# Autodesk Inventor assembly: Platform assembly
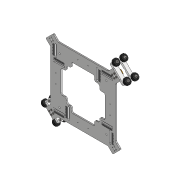
[picture p0: Inventor's stored thumbnail of the model, 180x180]
Saved by Autodesk Inventor 2020 (Build 240168000, 168)
## iProperties
Created: 2020-12-15
Part Number: Platform assembly
Document SubType Name: Assembly
Designer: ferrerx
Author: ferrerx
## Documents named in this file (4)
- C:\Users\ferrerx\Desktop\Prieto-Godino Lab\Drosophila Larvae Behavioural Device\Device design V3\Inventor Assembly\Platform assembly.iam
- C:\Users\ferrerx\Desktop\Prieto-Godino Lab\Drosophila Larvae Behavioural Device\Device design V3\Inventor Assembly\Light sources platform.ipt
- C:\Users\ferrerx\Desktop\Prieto-Godino Lab\Drosophila Larvae Behavioural Device\Device design V3\Inventor Assembly\Cart assembly.iam
- C:\Users\ferrerx\Documents\Inventor\Content Center Files\R2020\en-US\AS 1427(05)\AS 1427 - M3 x 25(5) II.ipt
## Components (11 placed, 3 different names)
1. Light sources platform:1 — Mate:1, Mate:2, Angle:1, Mate:3, Mate:4, Angle:2, Mate:6, Mate:7, Mate:8, Mate:9, Mate:10, Mate:11, Mate:12, Mate:13, Mate:14, Mate:15, Mate:16, Mate:17, Mate:18, Mate:19, Mate:20
2. Cart assembly:1 [sub-assembly] — Mate:1, Mate:2, Angle:1, Mate:5
3. Cart assembly:2 [sub-assembly] — Mate:3, Mate:4, Angle:2
4. AS 1427 H - Metric M3 x 25:1 — Mate:5, Mate:6
5. AS 1427 H - Metric M3 x 25:2 — Mate:7, Mate:19
6. AS 1427 H - Metric M3 x 25:3 — Mate:9, Mate:20
7. AS 1427 H - Metric M3 x 25:4 — Mate:8, Mate:18
8. AS 1427 H - Metric M3 x 25:5 — Mate:12, Mate:16
9. AS 1427 H - Metric M3 x 25:6 — Mate:10, Mate:17
10. AS 1427 H - Metric M3 x 25:7 — Mate:13, Mate:14
11. AS 1427 H - Metric M3 x 25:8 — Mate:11, Mate:15
## Relationships (22: Mate 20, Angle 2)
- Mate:1: Light sources platform:1 ↔ Cart assembly:1
- Mate:2: Light sources platform:1 ↔ Cart assembly:1
- Angle:1 (0 deg): Light sources platform:1 ↔ Cart assembly:1
- Mate:3: Light sources platform:1 ↔ Cart assembly:2
- Mate:4: Light sources platform:1 ↔ Cart assembly:2
- Angle:2 (0 deg): Light sources platform:1 ↔ Cart assembly:2
- Mate:5: Cart assembly:1 ↔ AS 1427 H - Metric M3 x 25:1
- Mate:6: Light sources platform:1 ↔ AS 1427 H - Metric M3 x 25:1
- Mate:7: Light sources platform:1 ↔ AS 1427 H - Metric M3 x 25:2
- Mate:8: Light sources platform:1 ↔ AS 1427 H - Metric M3 x 25:4
- Mate:9: Light sources platform:1 ↔ AS 1427 H - Metric M3 x 25:3
- Mate:10: Light sources platform:1 ↔ AS 1427 H - Metric M3 x 25:6
- Mate:11: Light sources platform:1 ↔ AS 1427 H - Metric M3 x 25:8
- Mate:12: Light sources platform:1 ↔ AS 1427 H - Metric M3 x 25:5
- Mate:13: Light sources platform:1 ↔ AS 1427 H - Metric M3 x 25:7
- Mate:14: Light sources platform:1 ↔ AS 1427 H - Metric M3 x 25:7
- Mate:15: Light sources platform:1 ↔ AS 1427 H - Metric M3 x 25:8
- Mate:16: Light sources platform:1 ↔ AS 1427 H - Metric M3 x 25:5
- Mate:17: Light sources platform:1 ↔ AS 1427 H - Metric M3 x 25:6
- Mate:18: Light sources platform:1 ↔ AS 1427 H - Metric M3 x 25:4
- Mate:19: Light sources platform:1 ↔ AS 1427 H - Metric M3 x 25:2
- Mate:20: Light sources platform:1 ↔ AS 1427 H - Metric M3 x 25:3
